# Autodesk Inventor assembly: Ensamble NotAFarmBot
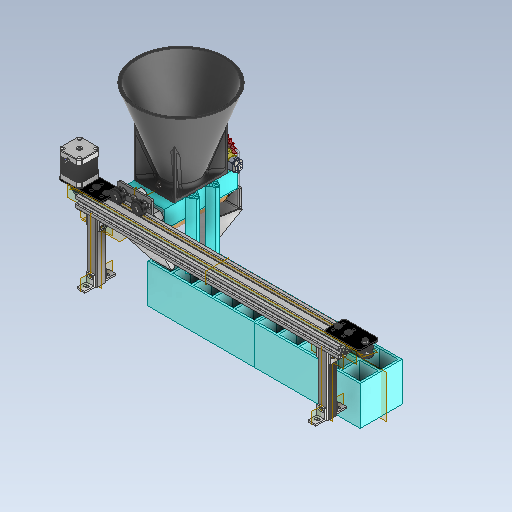
[picture p0: Inventor's stored thumbnail of the model, 512x512]
Saved by Autodesk Inventor 2020.3 (Build 243373000, 373)
## iProperties
Created: 2020-07-22
Part Number: Ensamble NotAFarmBot
Document SubType Name: Assembly
Designer: juanp
Mass: 2768.3 g
Surface Area: 9738.48 cm^2
Volume: 1823.12 cm^3
Density: 1.51844 g/cm^3
Author: juanp
## Documents named in this file (26)
- C:\Users\juanp\Desktop\ROBOCOL\Idea Final NAF\Ensamble NotAFarmBot.iam
- C:\Users\juanp\Desktop\ROBOCOL\Idea Final NAF\VSLOT 2040 Extrusion.ipt
- C:\Users\juanp\Desktop\ROBOCOL\Idea Final NAF\Double Tee Nut.ipt
- C:\Users\juanp\Desktop\ROBOCOL\Idea Final NAF\GT2_30T_5_6.ipt
- C:\Users\juanp\Desktop\ROBOCOL\Idea Final NAF\Idler Pulley Plate.ipt
- C:\Users\juanp\Desktop\ROBOCOL\Idea Final NAF\Motor Mount Plate Nema 17.ipt
- C:\Users\juanp\Desktop\ROBOCOL\Idea Final NAF\NEMA 17 simple\M1173041- NEMA 17.ipt
- C:\Users\juanp\Desktop\ROBOCOL\Idea Final NAF\Gantry\Inventor\20mm Gantry Set.iam
- C:\Users\juanp\Desktop\ROBOCOL\Idea Final NAF\3mm Spacer.ipt
- C:\Users\juanp\Desktop\ROBOCOL\Idea Final NAF\VSLOT Attachments\M5x25 low profile screw.ipt
- C:\Users\juanp\Desktop\ROBOCOL\Idea Final NAF\VSLOT Attachments\Ball Bearing 625 2RS 5x16x5.ipt
- C:\Users\juanp\Desktop\ROBOCOL\Idea Final NAF\VSLOT Attachments\1mm 5mm shim.ipt
- C:\Users\juanp\Desktop\ROBOCOL\Idea Final NAF\VSLOT Attachments\Nylon Spacer 1_8th.ipt
- C:\Users\juanp\Desktop\ROBOCOL\Idea Final NAF\VSLOT Attachments\idler pulley.ipt
- C:\Users\juanp\Desktop\ROBOCOL\Idea Final NAF\Gantry\Inventor\M5 Nylock.ipt
- C:\Users\juanp\Desktop\ROBOCOL\Idea Final NAF\VSLOT Attachments\M5x8 low profile screw.ipt
- C:\Users\juanp\Documents\Inventor\Content Center Files\R2020\en-US\ANSI B18.3.4M(1)\ANSI B18.3.4M - M3 x 0.5 x 8(2).ipt
- C:\Users\juanp\Desktop\ROBOCOL\Idea Final NAF\Contenedor Ensamblado.iam
- C:\Users\juanp\Desktop\ROBOCOL\Idea Final NAF\Dispensador\Ensamble Dispensador.iam
- C:\Users\juanp\Documents\Inventor\Content Center Files\R2020\en-US\ANSI B18.16.3M(2)\ANSI B18.16.3M - Property Class 5 and 10 - Metric M5 x 0.8 Metal Type.ipt
- C:\Users\juanp\Documents\Inventor\Content Center Files\R2020\en-US\ANSI B18.3.4M(2)\ANSI B18.3.4M - M5 x 0.8 x 12(1).ipt
- C:\Users\juanp\Documents\Inventor\Content Center Files\R2020\en-US\ANSI B18.3.4M(2)\ANSI B18.3.4M - M6 x 1 x 16(1).ipt
- C:\Users\juanp\Documents\Inventor\Content Center Files\R2020\en-US\ANSI B18.16.3M(2)\ANSI B18.16.3M - Property Class 5 and 10 - Metric M6 x 1 Metal Type.ipt
- C:\Users\juanp\Desktop\ROBOCOL\Idea Final NAF\ASTM A513 - 3_4 x 3_4 x 13_200 - 0.001.ipt
- C:\Users\juanp\Desktop\ROBOCOL\Idea Final NAF\ASTM A513 - 3_4 x 3_4 x 13_200 - 0.001_MIR.ipt
- C:\Users\juanp\Desktop\ROBOCOL\Idea Final NAF\VSLOT Attachments\L bracket single.ipt
## Components (40 placed, 25 different names)
1. VSLOT 2040 Extrusion:1 — Angle:5, Angle:6, Tangent:1, Tangent:2, Angle:7, Angle:8, Mate:57, Mate:58, Mate:77, Mate:78, Flush:63, Flush:64, Mate:79, Flush:65, Mate:85, Mate:86, Mate:87, Mate:88, Angle:16, Mate:98, Mate:99, Angle:18, Mate:100, Mate:101, Mate:109, Mate:112, Mate:114, Mate:116
2. Double Tee Nut:1 — Mate:98, Mate:99, Angle:18, Mate:100, Mate:106
3. Double Tee Nut:2 — Mate:85, Mate:86, Mate:87, Mate:93, Angle:16, Mate:94
4. GT2_30T_5_6:2 — Mate:35, Mate:107
5. Idler Pulley Plate:1 — Mate:88, Mate:89, Mate:90, Mate:91, Mate:92, Mate:95, Mate:96, Mate:97, Angle:17
6. Motor Mount Plate Nema 17:1 — Mate:12, Mate:13, Angle:4, Mate:42, Mate:43, Mate:52, Mate:53, Mate:54, Mate:55, Mate:56, Mate:101, Mate:102, Mate:103, Mate:104, Mate:105
7. M1173041- NEMA 17:1 — Mate:12, Mate:13, Angle:4, Mate:48, Mate:49, Mate:50, Mate:51, Mate:107
8. 20mm Gantry Set:1 [sub-assembly] — Angle:5, Angle:6, Tangent:1, Tangent:2, Mate:56, Mate:60, Mate:65, Mate:69, Mate:70, Mate:71, Mate:75, Mate:76
9. M5x25 low profile screw:1 — Mate:27, Mate:28, Mate:29, Mate:31, Mate:46, Mate:96
10. Ball Bearing 625 2RS 5x16x5:1 — Mate:22, Mate:23, Mate:24, Mate:26, Mate:32
11. Ball Bearing 625 2RS 5x16x5:2 — Mate:21, Mate:25, Mate:28
12. 1mm 5mm shim:1 — Mate:29, Mate:47, Mate:97
13. Nylon Spacer 1_8th:1 — Mate:23, Mate:24, Mate:25
14. idler pulley:1 — Mate:21, Mate:22, Mate:26, Mate:27, Mate:35
15. 3mm Spacer:1 — Mate:31, Mate:32, Mate:95
16. M5x8 low profile screw:1 — Mate:42, Mate:102, Mate:104
17. M5x8 low profile screw:2 — Mate:43, Mate:103, Mate:105, Mate:106
18. M5x8 low profile screw:3 — Mate:90, Mate:92, Mate:94
19. M5x8 low profile screw:4 — Mate:89, Mate:91, Mate:93
20. M5 Nylock:1 — Mate:46, Mate:47, Angle:17
21. Broached Hexagon Socket Button Head Cap Screw - Metric M3 x 0.5 x 8:1 — Mate:50, Mate:54
22. Broached Hexagon Socket Button Head Cap Screw - Metric M3 x 0.5 x 8:2 — Mate:51, Mate:55
23. Broached Hexagon Socket Button Head Cap Screw - Metric M3 x 0.5 x 8:3 — Mate:49, Mate:52
24. Broached Hexagon Socket Button Head Cap Screw - Metric M3 x 0.5 x 8:4 — Mate:48, Mate:53
25. Contenedor Ensamblado:1 [sub-assembly] — Angle:7, Angle:8, Mate:57, Mate:58, Angle:12, Flush:61, Mate:59, Mate:67, Mate:68, Flush:62
26. Ensamble Dispensador:1 [sub-assembly] — Angle:12, Flush:61, Mate:59, Mate:60, Angle:14, Mate:61, Mate:65, Mate:71, Angle:15, Mate:73
27. Prevailing Torque Type Hex Nut - Steel Metric Property Class 5 and 10 - Metric M5 x 0.8 Metal Type:1 — Angle:14, Mate:61, Mate:74
28. Forged Hexagon Socket Button Head Cap Screw - Metric M5 x 0.8 x 12:1 — Mate:74, Mate:75, Mate:76
29. Forged Hexagon Socket Button Head Cap Screw - Metric M6 x 1 x 16:1 — Mate:69, Mate:70, Mate:72
30. Prevailing Torque Type Hex Nut - Steel Metric Property Class 5 and 10 - Metric M6 x 1 Metal Type:1 — Mate:72, Angle:15, Mate:73
31. ASTM A513 - 3_4 x 3_4 x 13_200 - 0.001:1 — Mate:77, Mate:78, Flush:63, Mate:82, Mate:83, Flush:69, Flush:70, Flush:72, Mate:111, Flush:73, Mate:115, Flush:75
32. ASTM A513 - 3_4 x 3_4 x 13_200 - 0.001_MIR:1 — Flush:64, Mate:79, Flush:65, Mate:80, Flush:66, Mate:81, Mate:84, Mate:108, Mate:110, Mate:113, Flush:74
33. L bracket single:1 — Mate:81, Flush:67, Flush:68
34. L bracket single:2 — Mate:115, Mate:116, Flush:75
35. L bracket single:3 — Mate:83, Flush:70, Flush:71
36. L bracket single:4 — Mate:113, Mate:114, Flush:74
37. L bracket single:5 — Mate:108, Mate:109, Mate:110
38. L bracket single:6 — Mate:80, Flush:66, Flush:67, Flush:68, Mate:84
39. L bracket single:7 — Mate:111, Mate:112, Flush:73
40. L bracket single:8 — Mate:82, Flush:69, Flush:71, Flush:72
## Relationships (111: Mate 83, Flush 15, Angle 11, Tangent 2)
- Mate:12: Motor Mount Plate Nema 17:1 ↔ M1173041- NEMA 17:1
- Mate:13: Motor Mount Plate Nema 17:1 ↔ M1173041- NEMA 17:1
- Angle:4 (0 deg): Motor Mount Plate Nema 17:1 ↔ M1173041- NEMA 17:1
- Angle:5 (0 deg): VSLOT 2040 Extrusion:1 ↔ 20mm Gantry Set:1
- Angle:6 (0 deg): VSLOT 2040 Extrusion:1 ↔ 20mm Gantry Set:1
- Tangent:1: VSLOT 2040 Extrusion:1 ↔ 20mm Gantry Set:1
- Tangent:2: VSLOT 2040 Extrusion:1 ↔ 20mm Gantry Set:1
- Mate:21: Ball Bearing 625 2RS 5x16x5:2 ↔ idler pulley:1
- Mate:22: Ball Bearing 625 2RS 5x16x5:1 ↔ idler pulley:1
- Mate:23: Ball Bearing 625 2RS 5x16x5:1 ↔ Nylon Spacer 1_8th:1
- Mate:24: Ball Bearing 625 2RS 5x16x5:1 ↔ Nylon Spacer 1_8th:1
- Mate:25: Ball Bearing 625 2RS 5x16x5:2 ↔ Nylon Spacer 1_8th:1
- Mate:26: Ball Bearing 625 2RS 5x16x5:1 ↔ idler pulley:1
- Mate:27: M5x25 low profile screw:1 ↔ idler pulley:1
- Mate:28: M5x25 low profile screw:1 ↔ Ball Bearing 625 2RS 5x16x5:2
- Mate:29: M5x25 low profile screw:1 ↔ 1mm 5mm shim:1
- Mate:31: M5x25 low profile screw:1 ↔ 3mm Spacer:1
- Mate:32: Ball Bearing 625 2RS 5x16x5:1 ↔ 3mm Spacer:1
- Mate:35: GT2_30T_5_6:2 ↔ idler pulley:1
- Mate:42: Motor Mount Plate Nema 17:1 ↔ M5x8 low profile screw:1
- Mate:43: Motor Mount Plate Nema 17:1 ↔ M5x8 low profile screw:2
- Mate:46: M5x25 low profile screw:1 ↔ M5 Nylock:1
- Mate:47: 1mm 5mm shim:1 ↔ M5 Nylock:1
- Mate:48: M1173041- NEMA 17:1 ↔ Broached Hexagon Socket Button Head Cap Screw - Metric M3 x 0.5 x 8:4
- Mate:49: M1173041- NEMA 17:1 ↔ Broached Hexagon Socket Button Head Cap Screw - Metric M3 x 0.5 x 8:3
- Mate:50: M1173041- NEMA 17:1 ↔ Broached Hexagon Socket Button Head Cap Screw - Metric M3 x 0.5 x 8:1
- Mate:51: M1173041- NEMA 17:1 ↔ Broached Hexagon Socket Button Head Cap Screw - Metric M3 x 0.5 x 8:2
- Mate:52: Motor Mount Plate Nema 17:1 ↔ Broached Hexagon Socket Button Head Cap Screw - Metric M3 x 0.5 x 8:3
- Mate:53: Motor Mount Plate Nema 17:1 ↔ Broached Hexagon Socket Button Head Cap Screw - Metric M3 x 0.5 x 8:4
- Mate:54: Motor Mount Plate Nema 17:1 ↔ Broached Hexagon Socket Button Head Cap Screw - Metric M3 x 0.5 x 8:1
- Mate:55: Motor Mount Plate Nema 17:1 ↔ Broached Hexagon Socket Button Head Cap Screw - Metric M3 x 0.5 x 8:2
- Mate:56: Motor Mount Plate Nema 17:1 ↔ 20mm Gantry Set:1
- Angle:7 (0 deg): VSLOT 2040 Extrusion:1 ↔ Contenedor Ensamblado:1
- Angle:8 (0 deg): VSLOT 2040 Extrusion:1 ↔ Contenedor Ensamblado:1
- Mate:57: VSLOT 2040 Extrusion:1 ↔ Contenedor Ensamblado:1
- Mate:58: VSLOT 2040 Extrusion:1 ↔ Contenedor Ensamblado:1
- Angle:12 (0 deg): Contenedor Ensamblado:1 ↔ Ensamble Dispensador:1
- Flush:61: Contenedor Ensamblado:1 ↔ Ensamble Dispensador:1
- Mate:59 (5 mm): Contenedor Ensamblado:1 ↔ Ensamble Dispensador:1
- Mate:60: 20mm Gantry Set:1 ↔ Ensamble Dispensador:1
- Angle:14 (0 deg): Ensamble Dispensador:1 ↔ Prevailing Torque Type Hex Nut - Steel Metric Property Class 5 and 10 - Metric M5 x 0.8 Metal Type:1
- Mate:61: Ensamble Dispensador:1 ↔ Prevailing Torque Type Hex Nut - Steel Metric Property Class 5 and 10 - Metric M5 x 0.8 Metal Type:1
- Mate:65: 20mm Gantry Set:1 ↔ Ensamble Dispensador:1
- Mate:67: Contenedor Ensamblado:1
- Mate:68: Contenedor Ensamblado:1
- Flush:62: Contenedor Ensamblado:1
- Mate:69: 20mm Gantry Set:1 ↔ Forged Hexagon Socket Button Head Cap Screw - Metric M6 x 1 x 16:1
- Mate:70: 20mm Gantry Set:1 ↔ Forged Hexagon Socket Button Head Cap Screw - Metric M6 x 1 x 16:1
- Mate:71: 20mm Gantry Set:1 ↔ Ensamble Dispensador:1
- Mate:72: Forged Hexagon Socket Button Head Cap Screw - Metric M6 x 1 x 16:1 ↔ Prevailing Torque Type Hex Nut - Steel Metric Property Class 5 and 10 - Metric M6 x 1 Metal Type:1
- Angle:15 (0 deg): Ensamble Dispensador:1 ↔ Prevailing Torque Type Hex Nut - Steel Metric Property Class 5 and 10 - Metric M6 x 1 Metal Type:1
- Mate:73: Ensamble Dispensador:1 ↔ Prevailing Torque Type Hex Nut - Steel Metric Property Class 5 and 10 - Metric M6 x 1 Metal Type:1
- Mate:74: Prevailing Torque Type Hex Nut - Steel Metric Property Class 5 and 10 - Metric M5 x 0.8 Metal Type:1 ↔ Forged Hexagon Socket Button Head Cap Screw - Metric M5 x 0.8 x 12:1
- Mate:75: 20mm Gantry Set:1 ↔ Forged Hexagon Socket Button Head Cap Screw - Metric M5 x 0.8 x 12:1
- Mate:76: 20mm Gantry Set:1 ↔ Forged Hexagon Socket Button Head Cap Screw - Metric M5 x 0.8 x 12:1
- Mate:77: VSLOT 2040 Extrusion:1 ↔ ASTM A513 - 3_4 x 3_4 x 13_200 - 0.001:1
- Mate:78: VSLOT 2040 Extrusion:1 ↔ ASTM A513 - 3_4 x 3_4 x 13_200 - 0.001:1
- Flush:63 (20.95 mm): VSLOT 2040 Extrusion:1 ↔ ASTM A513 - 3_4 x 3_4 x 13_200 - 0.001:1
- Flush:64: VSLOT 2040 Extrusion:1 ↔ ASTM A513 - 3_4 x 3_4 x 13_200 - 0.001_MIR:1
- Mate:79: VSLOT 2040 Extrusion:1 ↔ ASTM A513 - 3_4 x 3_4 x 13_200 - 0.001_MIR:1
- Flush:65 (-20.95 mm): VSLOT 2040 Extrusion:1 ↔ ASTM A513 - 3_4 x 3_4 x 13_200 - 0.001_MIR:1
- Mate:80: ASTM A513 - 3_4 x 3_4 x 13_200 - 0.001_MIR:1 ↔ L bracket single:6
- Flush:66: ASTM A513 - 3_4 x 3_4 x 13_200 - 0.001_MIR:1 ↔ L bracket single:6
- Mate:81: ASTM A513 - 3_4 x 3_4 x 13_200 - 0.001_MIR:1 ↔ L bracket single:1
- Flush:67: L bracket single:1 ↔ L bracket single:6
- Flush:68: L bracket single:1 ↔ L bracket single:6
- Mate:82: ASTM A513 - 3_4 x 3_4 x 13_200 - 0.001:1 ↔ L bracket single:8
- Mate:83: ASTM A513 - 3_4 x 3_4 x 13_200 - 0.001:1 ↔ L bracket single:3
- Flush:69: ASTM A513 - 3_4 x 3_4 x 13_200 - 0.001:1 ↔ L bracket single:8
- Flush:70: ASTM A513 - 3_4 x 3_4 x 13_200 - 0.001:1 ↔ L bracket single:3
- Flush:71: L bracket single:3 ↔ L bracket single:8
- Mate:84: ASTM A513 - 3_4 x 3_4 x 13_200 - 0.001_MIR:1 ↔ L bracket single:6
- Flush:72: ASTM A513 - 3_4 x 3_4 x 13_200 - 0.001:1 ↔ L bracket single:8
- Mate:85: VSLOT 2040 Extrusion:1 ↔ Double Tee Nut:2
- Mate:86 (-10 mm): VSLOT 2040 Extrusion:1 ↔ Double Tee Nut:2
- Mate:87: VSLOT 2040 Extrusion:1 ↔ Double Tee Nut:2
- Mate:88: VSLOT 2040 Extrusion:1 ↔ Idler Pulley Plate:1
- Mate:89: Idler Pulley Plate:1 ↔ M5x8 low profile screw:4
- Mate:90: Idler Pulley Plate:1 ↔ M5x8 low profile screw:3
- Mate:91: Idler Pulley Plate:1 ↔ M5x8 low profile screw:4
- Mate:92: Idler Pulley Plate:1 ↔ M5x8 low profile screw:3
- Mate:93: Double Tee Nut:2 ↔ M5x8 low profile screw:4
- Angle:16 (180 deg): VSLOT 2040 Extrusion:1 ↔ Double Tee Nut:2
- Mate:94: Double Tee Nut:2 ↔ M5x8 low profile screw:3
- Mate:95: Idler Pulley Plate:1 ↔ 3mm Spacer:1
- Mate:96: Idler Pulley Plate:1 ↔ M5x25 low profile screw:1
- Mate:97: Idler Pulley Plate:1 ↔ 1mm 5mm shim:1
- Angle:17 (0 deg): Idler Pulley Plate:1 ↔ M5 Nylock:1
- Mate:98: VSLOT 2040 Extrusion:1 ↔ Double Tee Nut:1
- Mate:99: VSLOT 2040 Extrusion:1 ↔ Double Tee Nut:1
- Angle:18 (0 deg): VSLOT 2040 Extrusion:1 ↔ Double Tee Nut:1
- Mate:100 (-10 mm): VSLOT 2040 Extrusion:1 ↔ Double Tee Nut:1
- Mate:101: VSLOT 2040 Extrusion:1 ↔ Motor Mount Plate Nema 17:1
- Mate:102: Motor Mount Plate Nema 17:1 ↔ M5x8 low profile screw:1
- Mate:103: Motor Mount Plate Nema 17:1 ↔ M5x8 low profile screw:2
- Mate:104: Motor Mount Plate Nema 17:1 ↔ M5x8 low profile screw:1
- Mate:105: Motor Mount Plate Nema 17:1 ↔ M5x8 low profile screw:2
- Mate:106: Double Tee Nut:1 ↔ M5x8 low profile screw:2
- Mate:107: GT2_30T_5_6:2 ↔ M1173041- NEMA 17:1
- Mate:108: ASTM A513 - 3_4 x 3_4 x 13_200 - 0.001_MIR:1 ↔ L bracket single:5
- Mate:109: VSLOT 2040 Extrusion:1 ↔ L bracket single:5
- Mate:110: ASTM A513 - 3_4 x 3_4 x 13_200 - 0.001_MIR:1 ↔ L bracket single:5
- Mate:111: ASTM A513 - 3_4 x 3_4 x 13_200 - 0.001:1 ↔ L bracket single:7
- Mate:112: VSLOT 2040 Extrusion:1 ↔ L bracket single:7
- Flush:73: ASTM A513 - 3_4 x 3_4 x 13_200 - 0.001:1 ↔ L bracket single:7
- Mate:113: ASTM A513 - 3_4 x 3_4 x 13_200 - 0.001_MIR:1 ↔ L bracket single:4
- Mate:114: VSLOT 2040 Extrusion:1 ↔ L bracket single:4
- Flush:74: ASTM A513 - 3_4 x 3_4 x 13_200 - 0.001_MIR:1 ↔ L bracket single:4
- Mate:115: ASTM A513 - 3_4 x 3_4 x 13_200 - 0.001:1 ↔ L bracket single:2
- Mate:116: VSLOT 2040 Extrusion:1 ↔ L bracket single:2
- Flush:75: ASTM A513 - 3_4 x 3_4 x 13_200 - 0.001:1 ↔ L bracket single:2
